# Autodesk Inventor assembly: Cube (Sample)
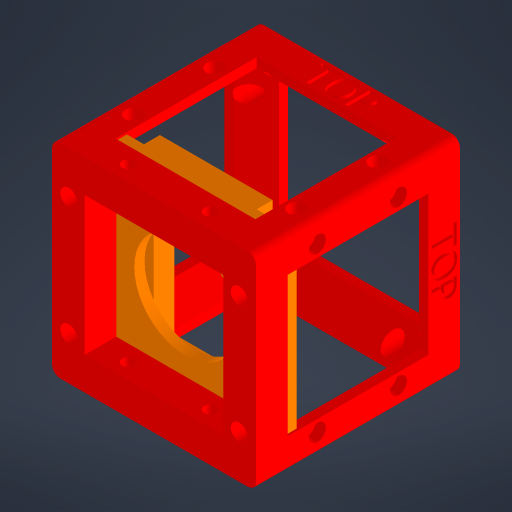
[picture p0: Inventor's stored thumbnail of the model, 512x512]
Saved by Autodesk Inventor 2023.4 (Build 274418000, 418)
## iProperties
Created: 2021-11-17
Part Number: Cube (Sample)
Document SubType Name: Assembly
Designer: xSibe
Author: xSibe
## Documents named in this file (4)
- C:\.Laptop\.Work\Projects\Project Protocube\Protocube\CAD, STL, OBJ Files\1 CAD\Sample\Cube (Sample).iam
- C:\.Laptop\.Work\Projects\Project Protocube\Protocube\CAD, STL, OBJ Files\1 CAD\Sample\Sample Clamp.ipt
- C:\.Laptop\.Work\Projects\Project Protocube\Protocube\CAD, STL, OBJ Files\1 CAD\Sample\Sample Holder.ipt
- C:\.Laptop\.Work\Projects\Project Protocube\Protocube\CAD, STL, OBJ Files\1 CAD\Cubes\Cube 1x1 V5.iam
## Components (3 placed, 3 different names)
1. Sample Holder:1 — Flush:3, Flush:4, Flush:5, Mate:1, Flush:6, Flush:7
2. Sample Clamp:1 — Flush:3, Flush:4, Flush:5
3. Cube 1x1 V5:1 [sub-assembly]
## Relationships (6: Flush 5, Mate 1)
- Flush:3: Sample Holder:1 ↔ Sample Clamp:1
- Flush:4: Sample Holder:1 ↔ Sample Clamp:1
- Flush:5: Sample Holder:1 ↔ Sample Clamp:1
- Mate:1: Sample Holder:1
- Flush:6: Sample Holder:1
- Flush:7: Sample Holder:1
